# Autodesk Inventor assembly: TopAssembly
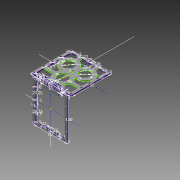
[picture p0: Inventor's stored thumbnail of the model, 180x180]
Saved by Autodesk Inventor 2014 SP1 (Build 180222100, 222)
## iProperties
Created: 2015-03-31
Part Number: TopAssembly
Document SubType Name: Assembly
Designer: Erin
Author: Erin
## Documents named in this file (4)
- C:\Users\Erin\Desktop\RDAS Base\TopAssembly.iam
- C:\Users\Erin\Desktop\RDAS Base\Side.ipt
- C:\Users\Erin\Desktop\RDAS Base\Top.ipt
- C:\Users\Erin\Desktop\RDAS Base\TopClip.ipt
## Components (3 placed, 3 different names)
1. Side:1 — Mate:1, Flush:1
2. Top:1 — Mate:1, Flush:1, Mate:2, Insert:1
3. TopClip:1 — Mate:2, Insert:1
## Relationships (4: Mate 2, Flush 1, Insert 1)
- Mate:1: Side:1 ↔ Top:1
- Flush:1: Side:1 ↔ Top:1
- Mate:2: Top:1 ↔ TopClip:1
- Insert:1: Top:1 ↔ TopClip:1
